# Autodesk Inventor assembly: base_final
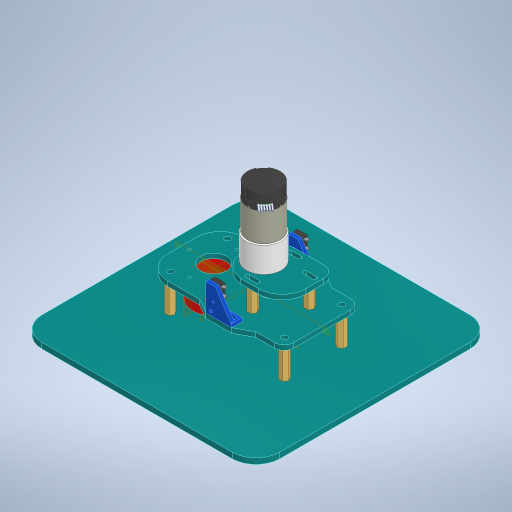
[picture p0: Inventor's stored thumbnail of the model, 512x512]
Saved by Autodesk Inventor 2024.3 (Build 283343000, 343)
## iProperties
Created: 2024-10-01
Part Number: base_final
Document SubType Name: Assembly
Designer: User
Author: User
## Documents named in this file (9)
- C:\Users\User\Documents\Universidad Octavo Semestre\Robotica Industrial\matlab\SCARA\mariana_scara_final\mariana_scara_final\base_final.iam
- C:\Users\User\Documents\Universidad Octavo Semestre\Robotica Industrial\matlab\SCARA\mariana_scara_final\mariana_scara_final\base.ipt
- C:\Users\User\Documents\Universidad Octavo Semestre\Robotica Industrial\matlab\SCARA\mariana_scara_final\mariana_scara_final\separador - copia.ipt
- C:\Users\User\Documents\Universidad Octavo Semestre\Robotica Industrial\matlab\SCARA\mariana_scara_final\mariana_scara_final\lamina_inferior.ipt
- C:\Users\User\Documents\Universidad Octavo Semestre\Robotica Industrial\matlab\SCARA\mariana_scara_final\mariana_scara_final\separador.ipt
- C:\Users\User\Documents\Universidad Octavo Semestre\Robotica Industrial\matlab\SCARA\mariana_scara_final\mariana_scara_final\BaseMotor1.iam
- C:\Users\User\Documents\Universidad Octavo Semestre\Robotica Industrial\matlab\SCARA\mariana_scara_final\mariana_scara_final\soporterto_damiento.ipt
- C:\Users\User\Documents\Universidad Octavo Semestre\Robotica Industrial\matlab\SCARA\mariana_scara_final\mariana_scara_final\final_carrera.iam
- C:\Users\User\Documents\Universidad Octavo Semestre\Robotica Industrial\matlab\SCARA\mariana_scara_final\mariana_scara_final\plea_peque.ipt
## Components (14 placed, 8 different names)
1. base:1 — Mate:1, Mate:2, Mate:3, Mate:4, Mate:5, Mate:6, Mate:7, Mate:8
2. separador - copia:1 — Mate:3, Mate:4, Mate:11
3. separador - copia:2 — Mate:1, Mate:2
4. separador - copia:3 — Mate:6, Mate:7, Mate:9, Mate:10
5. separador - copia:4 — Mate:5, Mate:8
6. lamina_inferior:1 — Mate:9, Mate:10, Mate:11, Mate:12, Mate:13, Mate:14, Mate:15, Mate:16, Mate:17, Mate:22, Mate:23, Mate:24, Flush:1, Mate:25, Mate:26, Flush:2, Mate:27, Mate:28
7. BaseMotor1:1 [sub-assembly] — Mate:18, Mate:19, Mate:20, Mate:21, Insert:1
8. separador:1 — Mate:12, Mate:15, Mate:19, Mate:21
9. separador:2 — Mate:13, Mate:16
10. separador:3 — Mate:14, Mate:17, Mate:18, Mate:20
11. soporterto_damiento:1 — Mate:22, Mate:23, Mate:24
12. final_carrera:1 [sub-assembly] — Flush:1, Mate:25, Mate:26
13. final_carrera:2 [sub-assembly] — Flush:2, Mate:27, Mate:28
14. plea_peque:1 — Insert:1
## Relationships (31: Mate 28, Flush 2, Insert 1)
- Mate:1: base:1 ↔ separador - copia:2
- Mate:2: base:1 ↔ separador - copia:2
- Mate:3: base:1 ↔ separador - copia:1
- Mate:4: base:1 ↔ separador - copia:1
- Mate:5: base:1 ↔ separador - copia:4
- Mate:6: base:1 ↔ separador - copia:3
- Mate:7: base:1 ↔ separador - copia:3
- Mate:8: base:1 ↔ separador - copia:4
- Mate:9: separador - copia:3 ↔ lamina_inferior:1
- Mate:10: separador - copia:3 ↔ lamina_inferior:1
- Mate:11: separador - copia:1 ↔ lamina_inferior:1
- Mate:12: lamina_inferior:1 ↔ separador:1
- Mate:13: lamina_inferior:1 ↔ separador:2
- Mate:14: lamina_inferior:1 ↔ separador:3
- Mate:15: lamina_inferior:1 ↔ separador:1
- Mate:16: lamina_inferior:1 ↔ separador:2
- Mate:17: lamina_inferior:1 ↔ separador:3
- Mate:18: BaseMotor1:1 ↔ separador:3
- Mate:19 (-1.9 mm): BaseMotor1:1 ↔ separador:1
- Mate:20 (5 mm): BaseMotor1:1 ↔ separador:3
- Mate:21 (5 mm): BaseMotor1:1 ↔ separador:1
- Mate:22: lamina_inferior:1 ↔ soporterto_damiento:1
- Mate:23: lamina_inferior:1 ↔ soporterto_damiento:1
- Mate:24: lamina_inferior:1 ↔ soporterto_damiento:1
- Flush:1: lamina_inferior:1 ↔ final_carrera:1
- Mate:25: lamina_inferior:1 ↔ final_carrera:1
- Mate:26: lamina_inferior:1 ↔ final_carrera:1
- Flush:2: lamina_inferior:1 ↔ final_carrera:2
- Mate:27: lamina_inferior:1 ↔ final_carrera:2
- Mate:28: lamina_inferior:1 ↔ final_carrera:2
- Insert:1: BaseMotor1:1 ↔ plea_peque:1
